# Autodesk Inventor assembly: main
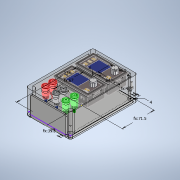
[picture p0: Inventor's stored thumbnail of the model, 180x180]
Saved by Autodesk Inventor 2022.1 (Build 261234020, 234B)
## iProperties
Created: 2022-02-06
Part Number: main
Document SubType Name: Assembly
Designer: kee
Mass: 279.206 g
Surface Area: 1857.64 cm^2
Volume: 229.168 cm^3
Density: 1.21834 g/cm^3
Author: kee
## Documents named in this file (7)
- C:\Users\logic\_workspace\2-ch-power-supply\hardware\casing\main.iam
- C:\Users\logic\_workspace\2-ch-power-supply\hardware\casing\standard_parts\DPS-5015\DPS_5015.iam
- C:\Users\logic\_workspace\2-ch-power-supply\hardware\casing\standard_parts\banana_jack\CT2236-0.iam
- C:\Users\logic\_workspace\2-ch-power-supply\hardware\casing\front_case.ipt
- C:\Users\logic\_workspace\2-ch-power-supply\hardware\casing\rear_case.ipt
- C:\Users\logic\_workspace\2-ch-power-supply\hardware\standard_parts\socket head cap screw 4762_din_EN ISO 4762 M3 x 10 - 10N.ipt
- C:\Users\logic\_workspace\2-ch-power-supply\hardware\casing\standard_parts\usb-c 20v v3\usb-c 20v v3.iam
## Components (15 placed, 7 different names)
1. DPS_5015:1 [sub-assembly] — Mate:1, Mate:3, Flush:5
2. DPS_5015:2 [sub-assembly] — Mate:1, Mate:2, Flush:5, Mate:4, Mate:5, Mate:6
3. CT2236-black:1 [sub-assembly] — Flush:4
4. CT2236-0:2 [sub-assembly]
5. CT2236-0:3 [sub-assembly]
6. CT2236-0:5 [sub-assembly] — Mate:2
7. CT2236-0:6 [sub-assembly]
8. CT2236-0:7 [sub-assembly]
9. front_case:1 — Mate:3, Mate:4, Mate:5, Mate:6, Mate:7, Flush:6
10. rear_case:1 — Mate:7, Flush:6
11. usb-c 20v v3:1 [sub-assembly]
12. socket head cap screw 4762_din_EN ISO 4762 M3 x 10 - 10N:1
13. socket head cap screw 4762_din_EN ISO 4762 M3 x 10 - 10N:2
14. socket head cap screw 4762_din_EN ISO 4762 M3 x 10 - 10N:3
15. socket head cap screw 4762_din_EN ISO 4762 M3 x 10 - 10N:4
## Relationships (10: Mate 7, Flush 3)
- Mate:1 (5 mm): DPS_5015:1 ↔ DPS_5015:2
- Flush:4: CT2236-black:1
- Mate:2: DPS_5015:2 ↔ CT2236-0:5
- Mate:3: DPS_5015:1 ↔ front_case:1
- Flush:5: DPS_5015:1 ↔ DPS_5015:2
- Mate:4: DPS_5015:2 ↔ front_case:1
- Mate:5: DPS_5015:2 ↔ front_case:1
- Mate:6: DPS_5015:2 ↔ front_case:1
- Mate:7: front_case:1 ↔ rear_case:1
- Flush:6: front_case:1 ↔ rear_case:1
